# Autodesk Inventor assembly: Simulation_module_2
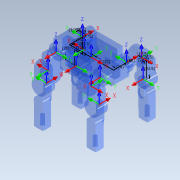
[picture p0: Inventor's stored thumbnail of the model, 180x180]
Saved by Autodesk Inventor 2020 (Build 240168000, 168)
## iProperties
Created: 2021-01-12
Part Number: Simulation_module_2
Document SubType Name: Assembly
Designer: DELL
Author: DELL
## Documents named in this file (5)
- F:\SoftRobot2.0\FlexipodHardware2.0\FlexipodHardware\Flexipod2.0\Cadquery_module\v4.0\Simulation_module.iam
- F:\SoftRobot2.0\FlexipodHardware2.0\FlexipodHardware\Flexipod2.0\Cadquery_module\v4.0\body.ipt
- F:\SoftRobot2.0\FlexipodHardware2.0\FlexipodHardware\Flexipod2.0\Cadquery_module\v4.0\hip.ipt
- F:\SoftRobot2.0\FlexipodHardware2.0\FlexipodHardware\Flexipod2.0\Cadquery_module\v4.0\thigh.ipt
- F:\SoftRobot2.0\FlexipodHardware2.0\FlexipodHardware\Flexipod2.0\Cadquery_module\v4.0\shank.ipt
## Components (13 placed, 4 different names)
1. body:1 — Mate:1, Mate:2, Flush:1, Flush:2, Flush:3, Angle:1, Angle:2, Angle:3, Mate:7, Mate:8, Angle:4, Angle:5, Mate:13, Mate:14, Angle:7, Mate:15, Mate:16, Angle:8
2. hip:1 — Mate:1, Mate:2, Angle:1, Mate:3, Mate:4
3. hip:2 — Mate:7, Mate:8, Angle:4, Mate:9, Mate:10
4. thigh:1 — Mate:3, Mate:4, Angle:2, Mate:5, Mate:6, Flush:4
5. thigh:2 — Mate:9, Mate:10, Angle:5, Mate:11, Mate:12, Angle:6
6. shank:1 — Mate:11, Mate:12, Angle:6
7. shank:2 — Mate:5, Mate:6, Angle:3, Flush:5
8. thigh:3 — Mate:13, Mate:14, Angle:7, Mate:17, Mate:18, Angle:9, Flush:7
9. thigh:4 — Mate:15, Mate:16, Angle:8, Mate:19, Mate:20, Angle:10
10. thigh:5 — Mate:17, Mate:18, Angle:9, Mate:23, Mate:24, Angle:12
11. thigh:6 — Mate:19, Mate:20, Angle:10, Mate:21, Mate:22, Angle:11
12. shank:3 — Mate:21, Mate:22, Angle:11
13. shank:4 — Mate:23, Mate:24, Angle:12, Flush:6
## Relationships (43: Mate 24, Angle 12, Flush 7)
- Mate:1: body:1 ↔ hip:1
- Mate:2: body:1 ↔ hip:1
- Flush:1: body:1
- Flush:2: body:1
- Flush:3: body:1
- Angle:1 (0 deg): body:1 ↔ hip:1
- Mate:3 (-10.5 mm): hip:1 ↔ thigh:1
- Mate:4: hip:1 ↔ thigh:1
- Angle:2 (0 deg): body:1 ↔ thigh:1
- Mate:5 (-9 mm): thigh:1 ↔ shank:2
- Mate:6: thigh:1 ↔ shank:2
- Angle:3 (0 deg): body:1 ↔ shank:2
- Mate:7: body:1 ↔ hip:2
- Mate:8: body:1 ↔ hip:2
- Angle:4 (0 deg): body:1 ↔ hip:2
- Mate:9 (-10.5 mm): hip:2 ↔ thigh:2
- Mate:10: hip:2 ↔ thigh:2
- Angle:5 (0 deg): body:1 ↔ thigh:2
- Mate:11 (-9 mm): thigh:2 ↔ shank:1
- Mate:12: thigh:2 ↔ shank:1
- Angle:6 (0 deg): thigh:2 ↔ shank:1
- Mate:13: body:1 ↔ thigh:3
- Mate:14: body:1 ↔ thigh:3
- Angle:7 (0 deg): body:1 ↔ thigh:3
- Mate:15: body:1 ↔ thigh:4
- Mate:16: body:1 ↔ thigh:4
- Angle:8 (0 deg): body:1 ↔ thigh:4
- Mate:17 (-9 mm): thigh:3 ↔ thigh:5
- Mate:18: thigh:3 ↔ thigh:5
- Angle:9 (0 deg): thigh:3 ↔ thigh:5
- Mate:19 (-9 mm): thigh:4 ↔ thigh:6
- Mate:20: thigh:4 ↔ thigh:6
- Angle:10 (0 deg): thigh:4 ↔ thigh:6
- Mate:21 (-9 mm): thigh:6 ↔ shank:3
- Mate:22: thigh:6 ↔ shank:3
- Angle:11 (0 deg): thigh:6 ↔ shank:3
- Mate:23 (-9 mm): thigh:5 ↔ shank:4
- Mate:24: thigh:5 ↔ shank:4
- Angle:12 (0 deg): thigh:5 ↔ shank:4
- Flush:4: thigh:1
- Flush:5: shank:2
- Flush:6: shank:4
- Flush:7: thigh:3
